# Autodesk Inventor assembly: bicon_m
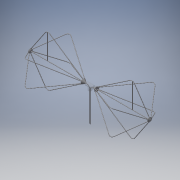
[picture p0: Inventor's stored thumbnail of the model, 180x180]
Saved by Autodesk Inventor 2019 (Build 230136000, 136)
## iProperties
Created: 2018-07-26
Part Number: bicon_m
Document SubType Name: Assembly
Designer: User
Author: User
## Documents named in this file (3)
- C:\Users\User\Documents\GitHub\darkRadio\3D Models\Bicon Antenna\bicon_m.iam
- C:\Users\User\Documents\GitHub\darkRadio\3D Models\Bicon Antenna\bicon_center_nate.ipt
- C:\Users\User\Documents\GitHub\darkRadio\3D Models\Bicon Antenna\bicon_arm_nate.ipt
## Components (3 placed, 2 different names)
1. bicon_center_nate:1 — Rigid:1, Rigid:2
2. bicon_arm_nate:1 — Rigid:1
3. bicon_arm_nate:2 — Rigid:2
## Relationships (2: WeldJoint 2)
- Rigid:1 [WeldJoint]: bicon_center_nate:1 ↔ bicon_arm_nate:1
- Rigid:2 [WeldJoint]: bicon_center_nate:1 ↔ bicon_arm_nate:2
